# Autodesk Inventor assembly: Почти готово_CPY
(part 2 of 2)
- Жесткий:1 [WeldJoint]: Втулка под палец_CPY:1 ↔ Крейцкопф_CPY:1
- Жесткий:3 [WeldJoint]: Втулка палец шатун_CPY:1 ↔ Втулка под палец_CPY:2
- Жесткий:2 [WeldJoint]: Крейцкопф_CPY:1 ↔ Втулка под палец_CPY:2
- Жесткий:5 [WeldJoint]: Крейцкопф_CPY:1 ↔ Башмак_CPY:2
- С поворотом:1 [RevoluteJoint]: Втулка под палец_CPY:1 ↔ Палец_CPY:1
- Жесткий:7 [WeldJoint]: Палец_CPY:1 ↔ Стопорное кольцо_CPY:1
- Жесткий:6 [WeldJoint]: Палец_CPY:1 ↔ Стопорное кольцо_CPY:2
- Жесткий:14 [WeldJoint]: Гайка шток-поршень_CPY:1 ↔ Кольцо поршень-шток верх_CPY:1
- Жесткий:13 [WeldJoint]: Верхняя часть поршня_CPY:1 ↔ Кольцо поршень-шток верх_CPY:1
- Жесткий:9 [WeldJoint]: Верхняя часть поршня_CPY:1 ↔ Кольцо поршня_CPY:1
- С поворотом:3 [RevoluteJoint]: Корпус дросселя_CPY:1 ↔ Корпус сальника_CPY:1
- Жесткий:16 [WeldJoint]: Втулка_CPY:1 ↔ Крышка цилиндра 1_CPY:1
- Жесткий:70 [WeldJoint] (-2 mm): Фонарь_CPY:1 ↔ Крышка цилиндра 2_CPY:1
- Жесткий:12 [WeldJoint]: Кольцо поршень-шток низ_CPY:1 ↔ Нижняя часть поршня_CPY:1
- Жесткий:8 [WeldJoint]: Верхняя часть поршня_CPY:1 ↔ Нижняя часть поршня_CPY:1
- Жесткий:21 [WeldJoint]: Нижняя часть поршня_CPY:1 ↔ Опорное кольцо_CPY:1
- Жесткий:27 [WeldJoint]: Кольцо сальника_CPY:1 ↔ Пружина сальника_CPY:1
- Жесткий:79 [WeldJoint]: Крышка цилиндра 2_CPY:1 ↔ Цилиндр2_CPY:1
- Жесткий:23 [WeldJoint] (1 mm): Крышка стакана_CPY:1 ↔ Цилиндр2_CPY:1
- Жесткий:15 [WeldJoint]: Втулка_CPY:1 ↔ Цилиндр2_CPY:1
- Жесткий:11 [WeldJoint]: Нижняя часть поршня_CPY:1 ↔ Кольцо поршня_CPY:2
- Цилиндрический:1 [CylindricalJoint]: Втулка_CPY:1 ↔ Кольцо поршня_CPY:3
- Жесткий:10 [WeldJoint]: Нижняя часть поршня_CPY:1 ↔ Кольцо поршня_CPY:3
- Жесткий:80 [WeldJoint] (-2 mm): Цилиндр2_CPY:1 ↔ Клапан1_CPY:1
- Жесткий:18 [WeldJoint]: Цилиндр2_CPY:1 ↔ Прокладка клапана_CPY:1
- Жесткий:81 [WeldJoint] (-22 mm): Цилиндр2_CPY:1 ↔ Стакан1_CPY:1
- Жесткий:20 [WeldJoint]: Верхняя часть поршня_CPY:1 ↔ Опорное кольцо_CPY:2
- Жесткий:26 [WeldJoint]: Корпус дросселя_CPY:1 ↔ Дроссельное кольцо_CPY:1
- Жесткий:25 [WeldJoint] (2 mm): Пружина дросселя_CPY:1 ↔ Дроссельное кольцо_CPY:1
- Жесткий:32 [WeldJoint]: Корпус сальника_CPY:1 ↔ Кольцо сальника_CPY:2
- Жесткий:31 [WeldJoint]: Кольцо сальника_CPY:1 ↔ Кольцо сальника_CPY:2
- Жесткий:28 [WeldJoint]: Кольцо сальника_CPY:2 ↔ Пружина сальника_CPY:2
- Жесткий:30 [WeldJoint]: Кольцо сальника_CPY:1 ↔ Кольцо сальника_CPY:3
- Жесткий:29 [WeldJoint]: Кольцо сальника_CPY:3 ↔ Пружина сальника_CPY:3
- Жесткий:57 [WeldJoint]: Корпус сальника_CPY:1 ↔ Корпус сальника_CPY:2
- Жесткий:33 [WeldJoint]: Кольцо сальника_CPY:4 ↔ Пружина сальника_CPY:4
- Жесткий:38 [WeldJoint]: Корпус сальника_CPY:2 ↔ Кольцо сальника_CPY:5
- Жесткий:37 [WeldJoint]: Кольцо сальника_CPY:4 ↔ Кольцо сальника_CPY:5
- Жесткий:34 [WeldJoint]: Кольцо сальника_CPY:5 ↔ Пружина сальника_CPY:5
- Жесткий:36 [WeldJoint]: Кольцо сальника_CPY:4 ↔ Кольцо сальника_CPY:6
- Жесткий:35 [WeldJoint]: Кольцо сальника_CPY:6 ↔ Пружина сальника_CPY:6
- Жесткий:58 [WeldJoint]: Корпус сальника_CPY:2 ↔ Корпус сальника_CPY:3
- Жесткий:39 [WeldJoint]: Кольцо сальника_CPY:7 ↔ Пружина сальника_CPY:7
- Жесткий:44 [WeldJoint]: Корпус сальника_CPY:3 ↔ Кольцо сальника_CPY:8
- Жесткий:43 [WeldJoint]: Кольцо сальника_CPY:7 ↔ Кольцо сальника_CPY:8
- Жесткий:40 [WeldJoint]: Кольцо сальника_CPY:8 ↔ Пружина сальника_CPY:8
- Жесткий:42 [WeldJoint]: Кольцо сальника_CPY:7 ↔ Кольцо сальника_CPY:9
- Жесткий:41 [WeldJoint]: Кольцо сальника_CPY:9 ↔ Пружина сальника_CPY:9
- Жесткий:59 [WeldJoint]: Корпус сальника_CPY:3 ↔ Корпус сальника_CPY:4
- Жесткий:45 [WeldJoint]: Кольцо сальника_CPY:10 ↔ Пружина сальника_CPY:10
- Жесткий:50 [WeldJoint]: Корпус сальника_CPY:4 ↔ Кольцо сальника_CPY:11
- Жесткий:49 [WeldJoint]: Кольцо сальника_CPY:10 ↔ Кольцо сальника_CPY:11
- Жесткий:46 [WeldJoint]: Кольцо сальника_CPY:11 ↔ Пружина сальника_CPY:11
- Жесткий:48 [WeldJoint]: Кольцо сальника_CPY:10 ↔ Кольцо сальника_CPY:12
- Жесткий:47 [WeldJoint]: Кольцо сальника_CPY:12 ↔ Пружина сальника_CPY:12
- Жесткий:60 [WeldJoint]: Корпус сальника_CPY:4 ↔ Корпус сальника_CPY:5
- Жесткий:51 [WeldJoint]: Кольцо сальника_CPY:13 ↔ Пружина сальника_CPY:13
- Жесткий:56 [WeldJoint]: Корпус сальника_CPY:5 ↔ Кольцо сальника_CPY:14
- Жесткий:55 [WeldJoint]: Кольцо сальника_CPY:13 ↔ Кольцо сальника_CPY:14
- Жесткий:52 [WeldJoint]: Кольцо сальника_CPY:14 ↔ Пружина сальника_CPY:14
- Жесткий:54 [WeldJoint]: Кольцо сальника_CPY:13 ↔ Кольцо сальника_CPY:15
- Жесткий:53 [WeldJoint]: Кольцо сальника_CPY:15 ↔ Пружина сальника_CPY:15
- Жесткий:62 [WeldJoint] (-1 mm): Корпус дросселя_CPY:1 ↔ Уплотнительное кольцо_CPY:1
- Жесткий:61 [WeldJoint] (1 mm): Крышка цилиндра 2_CPY:1 ↔ Уплотнительное кольцо_CPY:1
- Жесткий:63 [WeldJoint]: Кольцо сальника_CPY:16 ↔ Пружина сальника_CPY:16
- Жесткий:67 [WeldJoint]: Кольцо сальника_CPY:16 ↔ Кольцо сальника_CPY:17
- Жесткий:64 [WeldJoint]: Кольцо сальника_CPY:17 ↔ Пружина сальника_CPY:17
- Жесткий:66 [WeldJoint]: Кольцо сальника_CPY:16 ↔ Кольцо сальника_CPY:18
- Жесткий:65 [WeldJoint]: Кольцо сальника_CPY:18 ↔ Пружина сальника_CPY:18
- Жесткий:69 [WeldJoint]: Фонарь_CPY:1 ↔ Уплотнение фонарь_CPY:1
- Жесткий:77 [WeldJoint]: Корпус сальника_CPY:5 ↔ Корпус сальника_CPY:6
- Жесткий:71 [WeldJoint]: Кольцо сальника_CPY:19 ↔ Пружина сальника_CPY:19
- Жесткий:76 [WeldJoint]: Корпус сальника_CPY:6 ↔ Кольцо сальника_CPY:20
- Жесткий:75 [WeldJoint]: Кольцо сальника_CPY:19 ↔ Кольцо сальника_CPY:20
- Жесткий:72 [WeldJoint]: Кольцо сальника_CPY:20 ↔ Пружина сальника_CPY:20
- Жесткий:74 [WeldJoint]: Кольцо сальника_CPY:19 ↔ Кольцо сальника_CPY:21
- Жесткий:73 [WeldJoint]: Кольцо сальника_CPY:21 ↔ Пружина сальника_CPY:21
- Жесткий:78 [WeldJoint] (3 mm): Крышка цилиндра 2_CPY:1 ↔ Крышка сальников_CPY:1
- Жесткий:95 [WeldJoint]: Корпус сальника перегородка 1_CPY:1 ↔ Крышка перегородки11_CPY:1
- Жесткий:94 [WeldJoint]: Фонарь_CPY:1 ↔ Крышка перегородки11_CPY:1
- Жесткий:96 [WeldJoint]: Корпус сальника перегородка 1_CPY:1 ↔ Крышка перегородки12_CPY:1
- Жесткий:104 [WeldJoint]: Корпус маслосъемника_CPY:1 ↔ Крышка перегородки21_CPY:1
- Жесткий:103 [WeldJoint]: Кольцо сальника_CPY:17 ↔ Крышка перегородки21_CPY:1
- Жесткий:98 [WeldJoint]: Фонарь_CPY:1 ↔ Крышка перегородки21_CPY:1
- Жесткий:105 [WeldJoint]: Крышка перегородки21_CPY:1 ↔ Крышка перегородки22_CPY:1
- Жесткий:99 [WeldJoint] (-1 mm): Маслосъемная пружина_CPY:1 ↔ Маслосъемное кольцо_CPY:1
- Жесткий:97 [WeldJoint]: Фонарь_CPY:1 ↔ Придав перегородки1_CPY:1
- Жесткий:82 [WeldJoint]: Кольцо сальника_CPY:22 ↔ Пружина сальника_CPY:22
- Жесткий:87 [WeldJoint]: Корпус сальника перегородка 1_CPY:1 ↔ Кольцо сальника_CPY:23
- Жесткий:86 [WeldJoint]: Кольцо сальника_CPY:22 ↔ Кольцо сальника_CPY:23
- Жесткий:83 [WeldJoint]: Кольцо сальника_CPY:23 ↔ Пружина сальника_CPY:23
- Жесткий:85 [WeldJoint]: Кольцо сальника_CPY:22 ↔ Кольцо сальника_CPY:24
- Жесткий:84 [WeldJoint]: Кольцо сальника_CPY:24 ↔ Пружина сальника_CPY:24
- Жесткий:88 [WeldJoint]: Кольцо сальника_CPY:25 ↔ Пружина сальника_CPY:25
- Жесткий:93 [WeldJoint]: Корпус сальника перегородка 1_CPY:1 ↔ Кольцо сальника_CPY:26
- Жесткий:92 [WeldJoint]: Кольцо сальника_CPY:25 ↔ Кольцо сальника_CPY:26
- Жесткий:89 [WeldJoint]: Кольцо сальника_CPY:26 ↔ Пружина сальника_CPY:26
- Жесткий:91 [WeldJoint]: Кольцо сальника_CPY:25 ↔ Кольцо сальника_CPY:27
- Жесткий:90 [WeldJoint]: Кольцо сальника_CPY:27 ↔ Пружина сальника_CPY:27
- Жесткий:102 [WeldJoint]: Корпус маслосъемника_CPY:1 ↔ Маслосъемное кольцо_CPY:2
- Жесткий:101 [WeldJoint]: Маслосъемное кольцо_CPY:1 ↔ Маслосъемное кольцо_CPY:2
- Жесткий:100 [WeldJoint] (-1 mm): Маслосъемная пружина_CPY:2 ↔ Маслосъемное кольцо_CPY:2
- Жесткий:106 [WeldJoint]: Фонарь_CPY:1 ↔ Придав перегородки1_CPY:2
- Жесткий:110 [WeldJoint] (-3 mm): Гайка шток_CPY:1 ↔ Шток_CPY:1
- Жесткий:107 [WeldJoint] (4.75 mm): Гайка шток-поршень_CPY:1 ↔ Шток_CPY:1
- Жесткий:207 [WeldJoint]: Фланецгайка_CPY:1 ↔ Прокладка крейцкопф_CPY:1
- Жесткий:206 [WeldJoint]: Крейцкопф_CPY:1 ↔ Прокладка крейцкопф_CPY:1
- Жесткий:112 [WeldJoint]: Крышка цилиндра 1_CPY:1 ↔ Шайба  ГОСТ 11371-78 25:1
- Жесткий:113 [WeldJoint] (-8.75 mm): Шпилька ГОСТ 22038-76 M24-6g×70:1 ↔ Гайка ГОСТ 15524-70 M24:1
- Жесткий:111 [WeldJoint]: Цилиндр2_CPY:1 ↔ Шпилька ГОСТ 22038-76 M24-6g×70:1
- Жесткий:114 [WeldJoint] (-8.75 mm): Шпилька ГОСТ 22038-76 M24-6g×70:2 ↔ Гайка ГОСТ 15524-70 M24:2
- Жесткий:116 [WeldJoint] (-2 mm): Цилиндр2_CPY:1 ↔ Клапан1_CPY:2
- Жесткий:115 [WeldJoint]: Цилиндр2_CPY:1 ↔ Прокладка клапана_CPY:2
- Жесткий:117 [WeldJoint] (-22 mm): Цилиндр2_CPY:1 ↔ Стакан1_CPY:2
- Жесткий:118 [WeldJoint] (1 mm): Цилиндр2_CPY:1 ↔ Крышка стакана_CPY:2
- Жесткий:119 [WeldJoint] (-1 mm): Цилиндр2_CPY:1 ↔ Шпилька ГОСТ 22034-76 M20-6g×50:1
- Жесткий:121 [WeldJoint] (-2.5 mm): Гайка ГОСТ 15521-70 M20:1 ↔ Шпилька ГОСТ 22034-76 M20-6g×50:1
- Жесткий:120 [WeldJoint] (-20 mm): Шпилька ГОСТ 22034-76 M20-6g×50:1 ↔ Шайба ГОСТ 10450-78 19:1
- Жесткий:122 [WeldJoint]: Цилиндр2_CPY:1 ↔ Шпилька ГОСТ 22034-76 M20-6g×50:2
- Жесткий:124 [WeldJoint] (-2.25 mm): Шпилька ГОСТ 22034-76 M20-6g×50:2 ↔ Гайка ГОСТ 15521-70 M20:2
- Жесткий:123 [WeldJoint] (-20 mm): Шпилька ГОСТ 22034-76 M20-6g×50:2 ↔ Шайба ГОСТ 10450-78 19:2
- Жесткий:127 [WeldJoint] (-2 mm): Фонарь_CPY:1 ↔ Гайка ГОСТ 15524-70 M20:1
- Жесткий:126 [WeldJoint] (-32 mm): Шпилька ГОСТ 22038-76 M20-6g×85:1 ↔ Шайба ГОСТ 10450-78 21:1
- Жесткий:125 [WeldJoint]: Крышка цилиндра 2_CPY:1 ↔ Шпилька ГОСТ 22038-76 M20-6g×85:1
- Жесткий:130 [WeldJoint]: Крышка перегородки22_CPY:1 ↔ Шайба  ГОСТ 11371-78 13:2
- Жесткий:134 [WeldJoint]: Придав перегородки1_CPY:1 ↔ Шайба  ГОСТ 11371-78 13:4
- Жесткий:128 [WeldJoint]: Крышка перегородки12_CPY:1 ↔ Шайба  ГОСТ 11371-78 13:1
- Жесткий:135 [WeldJoint]: Шайба  ГОСТ 11371-78 13:4 ↔ Винт ГОСТ 11738-84 M 10x25:2
- Жесткий:133 [WeldJoint]: Винт ГОСТ 11738-84 M 10x25:1 ↔ Шайба  ГОСТ 11371-78 13:3
- Жесткий:132 [WeldJoint]: Придав перегородки1_CPY:2 ↔ Шайба  ГОСТ 11371-78 13:3
- Жесткий:129 [WeldJoint]: Винт ГОСТ 11738-84 M 10x35:1 ↔ Шайба  ГОСТ 11371-78 13:1
- Жесткий:131 [WeldJoint]: Винт ГОСТ 11738-84 M 10x30:1 ↔ Шайба  ГОСТ 11371-78 13:2
- Жесткий:138 [WeldJoint] (-38 mm): Шпилька ГОСТ 22038-76 M24-6g×80:1 ↔ Гайка ГОСТ 15524-70 M24:18
- Жесткий:137 [WeldJoint] (-38 mm): Шпилька ГОСТ 22038-76 M24-6g×80:1 ↔ Шайба  ГОСТ 11371-78 28:1
- Жесткий:140 [WeldJoint] (-38 mm): Шпилька ГОСТ 22038-76 M24-6g×80:2 ↔ Гайка ГОСТ 15524-70 M24:19
- Жесткий:163 [WeldJoint]: Фонарь_CPY:1 ↔ Шайба  ГОСТ 11371-78 28:2
- Жесткий:139 [WeldJoint] (-38 mm): Шпилька ГОСТ 22038-76 M24-6g×80:2 ↔ Шайба  ГОСТ 11371-78 28:2
- Жесткий:142 [WeldJoint] (-38 mm): Шпилька ГОСТ 22038-76 M24-6g×80:3 ↔ Гайка ГОСТ 15524-70 M24:20
- Жесткий:165 [WeldJoint]: Фонарь_CPY:1 ↔ Шайба  ГОСТ 11371-78 28:3
- Жесткий:141 [WeldJoint] (-38 mm): Шпилька ГОСТ 22038-76 M24-6g×80:3 ↔ Шайба  ГОСТ 11371-78 28:3
- Жесткий:144 [WeldJoint] (-38 mm): Шпилька ГОСТ 22038-76 M24-6g×80:4 ↔ Гайка ГОСТ 15524-70 M24:21
- Жесткий:166 [WeldJoint]: Фонарь_CPY:1 ↔ Шайба  ГОСТ 11371-78 28:4
- Жесткий:143 [WeldJoint] (-38 mm): Шпилька ГОСТ 22038-76 M24-6g×80:4 ↔ Шайба  ГОСТ 11371-78 28:4
- Жесткий:146 [WeldJoint] (-38 mm): Шпилька ГОСТ 22038-76 M24-6g×80:5 ↔ Гайка ГОСТ 15524-70 M24:22
- Жесткий:164 [WeldJoint]: Фонарь_CPY:1 ↔ Шайба  ГОСТ 11371-78 28:5
- Жесткий:145 [WeldJoint] (-38 mm): Шпилька ГОСТ 22038-76 M24-6g×80:5 ↔ Шайба  ГОСТ 11371-78 28:5
- Жесткий:148 [WeldJoint] (-38 mm): Шпилька ГОСТ 22038-76 M24-6g×80:6 ↔ Гайка ГОСТ 15524-70 M24:23
- Жесткий:171 [WeldJoint]: Фонарь_CPY:1 ↔ Шайба  ГОСТ 11371-78 28:6
- Жесткий:147 [WeldJoint] (-38 mm): Шпилька ГОСТ 22038-76 M24-6g×80:6 ↔ Шайба  ГОСТ 11371-78 28:6
- Жесткий:150 [WeldJoint] (-38 mm): Шпилька ГОСТ 22038-76 M24-6g×80:7 ↔ Гайка ГОСТ 15524-70 M24:24
- Жесткий:173 [WeldJoint]: Фонарь_CPY:1 ↔ Шайба  ГОСТ 11371-78 28:7
- Жесткий:149 [WeldJoint] (-38 mm): Шпилька ГОСТ 22038-76 M24-6g×80:7 ↔ Шайба  ГОСТ 11371-78 28:7
- Жесткий:152 [WeldJoint] (-38 mm): Шпилька ГОСТ 22038-76 M24-6g×80:8 ↔ Гайка ГОСТ 15524-70 M24:25
- Жесткий:174 [WeldJoint]: Фонарь_CPY:1 ↔ Шайба  ГОСТ 11371-78 28:8
- Жесткий:151 [WeldJoint] (-38 mm): Шпилька ГОСТ 22038-76 M24-6g×80:8 ↔ Шайба  ГОСТ 11371-78 28:8
- Жесткий:154 [WeldJoint] (-38 mm): Шпилька ГОСТ 22038-76 M24-6g×80:9 ↔ Гайка ГОСТ 15524-70 M24:26
- Жесткий:172 [WeldJoint]: Фонарь_CPY:1 ↔ Шайба  ГОСТ 11371-78 28:9
- Жесткий:153 [WeldJoint] (-38 mm): Шпилька ГОСТ 22038-76 M24-6g×80:9 ↔ Шайба  ГОСТ 11371-78 28:9
- Жесткий:156 [WeldJoint] (-38 mm): Шпилька ГОСТ 22038-76 M24-6g×80:10 ↔ Гайка ГОСТ 15524-70 M24:27
- Жесткий:169 [WeldJoint]: Фонарь_CPY:1 ↔ Шайба  ГОСТ 11371-78 28:10
- Жесткий:155 [WeldJoint] (-38 mm): Шпилька ГОСТ 22038-76 M24-6g×80:10 ↔ Шайба  ГОСТ 11371-78 28:10
- Жесткий:158 [WeldJoint] (-38 mm): Шпилька ГОСТ 22038-76 M24-6g×80:11 ↔ Гайка ГОСТ 15524-70 M24:28
- Жесткий:167 [WeldJoint]: Фонарь_CPY:1 ↔ Шайба  ГОСТ 11371-78 28:11
- Жесткий:157 [WeldJoint] (-38 mm): Шпилька ГОСТ 22038-76 M24-6g×80:11 ↔ Шайба  ГОСТ 11371-78 28:11
- Жесткий:160 [WeldJoint] (-38 mm): Шпилька ГОСТ 22038-76 M24-6g×80:12 ↔ Гайка ГОСТ 15524-70 M24:29
- Жесткий:170 [WeldJoint]: Фонарь_CPY:1 ↔ Шайба  ГОСТ 11371-78 28:12
- Жесткий:159 [WeldJoint] (-38 mm): Шпилька ГОСТ 22038-76 M24-6g×80:12 ↔ Шайба  ГОСТ 11371-78 28:12
- Жесткий:162 [WeldJoint] (-38 mm): Шпилька ГОСТ 22038-76 M24-6g×80:13 ↔ Гайка ГОСТ 15524-70 M24:30
- Жесткий:168 [WeldJoint]: Фонарь_CPY:1 ↔ Шайба  ГОСТ 11371-78 28:13
- Жесткий:161 [WeldJoint] (-38 mm): Шпилька ГОСТ 22038-76 M24-6g×80:13 ↔ Шайба  ГОСТ 11371-78 28:13
- Жесткий:176 [WeldJoint] (-38 mm): Шпилька ГОСТ 22038-76 M24-6g×80:14 ↔ Гайка ГОСТ 15524-70 M24:31
- Жесткий:192 [WeldJoint]: Фонарь_CPY:1 ↔ Шайба  ГОСТ 11371-78 28:14
- Жесткий:175 [WeldJoint] (-38 mm): Шпилька ГОСТ 22038-76 M24-6g×80:14 ↔ Шайба  ГОСТ 11371-78 28:14
- Жесткий:178 [WeldJoint] (-38 mm): Шпилька ГОСТ 22038-76 M24-6g×80:15 ↔ Гайка ГОСТ 15524-70 M24:32
- Жесткий:197 [WeldJoint]: Фонарь_CPY:1 ↔ Шайба  ГОСТ 11371-78 28:15
- Жесткий:177 [WeldJoint] (-38 mm): Шпилька ГОСТ 22038-76 M24-6g×80:15 ↔ Шайба  ГОСТ 11371-78 28:15
- Жесткий:180 [WeldJoint] (-38 mm): Шпилька ГОСТ 22038-76 M24-6g×80:16 ↔ Гайка ГОСТ 15524-70 M24:33
- Жесткий:191 [WeldJoint]: Фонарь_CPY:1 ↔ Шайба  ГОСТ 11371-78 28:16
- Жесткий:179 [WeldJoint] (-38 mm): Шпилька ГОСТ 22038-76 M24-6g×80:16 ↔ Шайба  ГОСТ 11371-78 28:16
- Жесткий:184 [WeldJoint] (-38 mm): Шпилька ГОСТ 22038-76 M24-6g×80:17 ↔ Гайка ГОСТ 15524-70 M24:34
- Жесткий:196 [WeldJoint]: Фонарь_CPY:1 ↔ Шайба  ГОСТ 11371-78 28:17
- Жесткий:183 [WeldJoint] (-38 mm): Шпилька ГОСТ 22038-76 M24-6g×80:17 ↔ Шайба  ГОСТ 11371-78 28:17
- Жесткий:186 [WeldJoint] (-38 mm): Шпилька ГОСТ 22038-76 M24-6g×80:18 ↔ Гайка ГОСТ 15524-70 M24:35
- Жесткий:194 [WeldJoint]: Фонарь_CPY:1 ↔ Шайба  ГОСТ 11371-78 28:18
- Жесткий:185 [WeldJoint] (-38 mm): Шпилька ГОСТ 22038-76 M24-6g×80:18 ↔ Шайба  ГОСТ 11371-78 28:18
- Жесткий:188 [WeldJoint] (-38 mm): Шпилька ГОСТ 22038-76 M24-6g×80:19 ↔ Гайка ГОСТ 15524-70 M24:36
- Жесткий:193 [WeldJoint]: Фонарь_CPY:1 ↔ Шайба  ГОСТ 11371-78 28:19
- Жесткий:187 [WeldJoint] (-38 mm): Шпилька ГОСТ 22038-76 M24-6g×80:19 ↔ Шайба  ГОСТ 11371-78 28:19
- Жесткий:190 [WeldJoint] (-38 mm): Шпилька ГОСТ 22038-76 M24-6g×80:20 ↔ Гайка ГОСТ 15524-70 M24:37
- Жесткий:195 [WeldJoint]: Фонарь_CPY:1 ↔ Шайба  ГОСТ 11371-78 28:20
- Жесткий:189 [WeldJoint] (-38 mm): Шпилька ГОСТ 22038-76 M24-6g×80:20 ↔ Шайба  ГОСТ 11371-78 28:20
- Жесткий:198 [WeldJoint] (-2.5 mm): Гайка ГОСТ 15521-70 M20:3 ↔ Шпилька ГОСТ 22034-76 M20-6g×50:3
- Жесткий:199 [WeldJoint] (-20 mm): Шпилька ГОСТ 22034-76 M20-6g×50:3 ↔ Шайба ГОСТ 10450-78 19:3
- Жесткий:200 [WeldJoint] (-2.25 mm): Шпилька ГОСТ 22034-76 M20-6g×50:4 ↔ Гайка ГОСТ 15521-70 M20:4
- Жесткий:201 [WeldJoint] (-20 mm): Шпилька ГОСТ 22034-76 M20-6g×50:4 ↔ Шайба ГОСТ 10450-78 19:4
- Жесткий:208 [WeldJoint]: Крейцкопф_CPY:1 ↔ Шпилька ГОСТ 22038-76 M20-6g×85:2
- Жесткий:209 [WeldJoint]: Крейцкопф_CPY:1 ↔ Шпилька ГОСТ 22038-76 M20-6g×85:3
- Жесткий:211 [WeldJoint] (-26 mm): Шпилька ГОСТ 22038-76 M20-6g×85:2 ↔ Гайка ГОСТ 15524-70 M20:2
- Жесткий:210 [WeldJoint] (-26 mm): Шпилька ГОСТ 22038-76 M20-6g×85:2 ↔ Шайба  ГОСТ 11371-78 23:1
- Жесткий:213 [WeldJoint] (-2 mm): Шпилька ГОСТ 22038-76 M20-6g×85:3 ↔ Гайка ГОСТ 15524-70 M20:3
- Жесткий:212 [WeldJoint] (-26 mm): Шпилька ГОСТ 22038-76 M20-6g×85:3 ↔ Шайба  ГОСТ 11371-78 23:2
- Жесткий:404 [WeldJoint] (298.75 mm): Шток_CPY:1 ↔ Маслоотражательное кольцо_CPY:1
- Заподлицо:9 [Flush]: Фонарь_CPY:1 ↔ Крышка фонаря 1:1
- Заподлицо:10 [Flush]: Фонарь_CPY:1 ↔ Крышка фонаря 1:1
- Заподлицо:11 [Flush]: Фонарь_CPY:1 ↔ Крышка фонаря 2:1
- Заподлицо:12 [Flush]: Фонарь_CPY:1 ↔ Крышка фонаря 2:1
- Жесткий:395 [WeldJoint]: Крышка фонаря 1:1 ↔ Болт ГОСТ Р 50274-92 M8-6g×16-F:101
- Жесткий:396 [WeldJoint]: Крышка фонаря 1:1 ↔ Болт ГОСТ Р 50274-92 M8-6g×16-F:105
- Жесткий:397 [WeldJoint]: Крышка фонаря 1:1 ↔ Болт ГОСТ Р 50274-92 M8-6g×16-F:104
- Жесткий:398 [WeldJoint]: Крышка фонаря 1:1 ↔ Болт ГОСТ Р 50274-92 M8-6g×16-F:106
- Жесткий:399 [WeldJoint]: Крышка фонаря 1:1 ↔ Болт ГОСТ Р 50274-92 M8-6g×16-F:119
- Жесткий:400 [WeldJoint]: Крышка фонаря 1:1 ↔ Болт ГОСТ Р 50274-92 M8-6g×16-F:65
- Жесткий:401 [WeldJoint]: Крышка фонаря 1:1 ↔ Болт ГОСТ Р 50274-92 M8-6g×16-F:123
- Жесткий:402 [WeldJoint]: Крышка фонаря 1:1 ↔ Болт ГОСТ Р 50274-92 M8-6g×16-F:107
- Жесткий:403 [WeldJoint]: Крышка фонаря 1:1 ↔ Болт ГОСТ Р 50274-92 M8-6g×16-F:110
- Жесткий:404 [WeldJoint]: Крышка фонаря 1:1 ↔ Болт ГОСТ Р 50274-92 M8-6g×16-F:108
- Жесткий:405 [WeldJoint]: Крышка фонаря 1:1 ↔ Болт ГОСТ Р 50274-92 M8-6g×16-F:114
- Жесткий:406 [WeldJoint]: Крышка фонаря 1:1 ↔ Болт ГОСТ Р 50274-92 M8-6g×16-F:102
- С поворотом:3 [RevoluteJoint]: Крышка фонаря 2:1 ↔ Болт ГОСТ Р 50274-92 M8-6g×16-F:69
- С поворотом:4 [RevoluteJoint]: Крышка фонаря 2:1 ↔ Болт ГОСТ Р 50274-92 M8-6g×16-F:70
- С поворотом:5 [RevoluteJoint]: Крышка фонаря 2:1 ↔ Болт ГОСТ Р 50274-92 M8-6g×16-F:83
- Жесткий:407 [WeldJoint]: Крышка фонаря 2:1 ↔ Болт ГОСТ Р 50274-92 M8-6g×16-F:95
- Жесткий:408 [WeldJoint]: Крышка фонаря 2:1 ↔ Болт ГОСТ Р 50274-92 M8-6g×16-F:92
- Жесткий:409 [WeldJoint]: Крышка фонаря 2:1 ↔ Болт ГОСТ Р 50274-92 M8-6g×16-F:87
- Жесткий:410 [WeldJoint]: Крышка фонаря 2:1 ↔ Болт ГОСТ Р 50274-92 M8-6g×16-F:71
- Жесткий:411 [WeldJoint]: Крышка фонаря 2:1 ↔ Болт ГОСТ Р 50274-92 M8-6g×16-F:115
- Жесткий:412 [WeldJoint]: Крышка фонаря 2:1 ↔ Болт ГОСТ Р 50274-92 M8-6g×16-F:124
- Жесткий:413 [WeldJoint]: Крышка фонаря 2:1 ↔ Болт ГОСТ Р 50274-92 M8-6g×16-F:128
- Жесткий:414 [WeldJoint]: Крышка фонаря 2:1 ↔ Болт ГОСТ Р 50274-92 M8-6g×16-F:77
- Жесткий:415 [WeldJoint]: Крышка фонаря 2:1 ↔ Болт ГОСТ Р 50274-92 M8-6g×16-F:74
- Жесткий:416 [WeldJoint]: Крышка фонаря 2:1 ↔ Болт ГОСТ Р 50274-92 M8-6g×16-F:72
- Жесткий:417 [WeldJoint]: Крышка фонаря 2:1 ↔ Болт ГОСТ Р 50274-92 M8-6g×16-F:78
- Жесткий:418 [WeldJoint]: Крышка фонаря 2:1 ↔ Болт ГОСТ Р 50274-92 M8-6g×16-F:132
- Жесткий:419 [WeldJoint]: Крышка фонаря 2:1 ↔ Болт ГОСТ Р 50274-92 M8-6g×16-F:76
- Жесткий:420 [WeldJoint]: Крышка фонаря 2:1 ↔ Болт ГОСТ Р 50274-92 M8-6g×16-F:88
- Жесткий:421 [WeldJoint]: Крышка фонаря 2:1 ↔ Болт ГОСТ Р 50274-92 M8-6g×16-F:79
- Жесткий:422 [WeldJoint]: Крышка фонаря 2:1 ↔ Болт ГОСТ Р 50274-92 M8-6g×16-F:82
- Жесткий:423 [WeldJoint]: Крышка фонаря 2:1 ↔ Болт ГОСТ Р 50274-92 M8-6g×16-F:89
- Жесткий:424 [WeldJoint]: Крышка фонаря 2:1 ↔ Болт ГОСТ Р 50274-92 M8-6g×16-F:66
- Жесткий:425 [WeldJoint]: Крышка фонаря 2:1 ↔ Болт ГОСТ Р 50274-92 M8-6g×16-F:96
- Жесткий:426 [WeldJoint]: Крышка фонаря 2:1 ↔ Болт ГОСТ Р 50274-92 M8-6g×16-F:118
- Жесткий:427 [WeldJoint]: Крышка фонаря 2:1 ↔ Болт ГОСТ Р 50274-92 M8-6g×16-F:80
- Жесткий:428 [WeldJoint]: Крышка фонаря 1_MIR1:1 ↔ Болт ГОСТ Р 50274-92 M8-6g×16-F:133
- Жесткий:429 [WeldJoint]: Крышка фонаря 2_MIR1:1 ↔ Болт ГОСТ Р 50274-92 M8-6g×16-F:134
- С поворотом:6 [RevoluteJoint]: Крышка фонаря 2_MIR1:1 ↔ Болт ГОСТ Р 50274-92 M8-6g×16-F:135
- С поворотом:7 [RevoluteJoint]: Крышка фонаря 2_MIR1:1 ↔ Болт ГОСТ Р 50274-92 M8-6g×16-F:136
- Жесткий:430 [WeldJoint]: Крышка фонаря 2_MIR1:1 ↔ Болт ГОСТ Р 50274-92 M8-6g×16-F:137
- Жесткий:431 [WeldJoint]: Крышка фонаря 2_MIR1:1 ↔ Болт ГОСТ Р 50274-92 M8-6g×16-F:138
- Жесткий:432 [WeldJoint]: Крышка фонаря 2_MIR1:1 ↔ Болт ГОСТ Р 50274-92 M8-6g×16-F:139
- Жесткий:433 [WeldJoint]: Крышка фонаря 2_MIR1:1 ↔ Болт ГОСТ Р 50274-92 M8-6g×16-F:140
- Жесткий:434 [WeldJoint]: Крышка фонаря 2_MIR1:1 ↔ Болт ГОСТ Р 50274-92 M8-6g×16-F:141
- Жесткий:435 [WeldJoint]: Крышка фонаря 2_MIR1:1 ↔ Болт ГОСТ Р 50274-92 M8-6g×16-F:142
- Жесткий:436 [WeldJoint]: Крышка фонаря 2_MIR1:1 ↔ Болт ГОСТ Р 50274-92 M8-6g×16-F:143
- Жесткий:437 [WeldJoint]: Крышка фонаря 2_MIR1:1 ↔ Болт ГОСТ Р 50274-92 M8-6g×16-F:144
- Жесткий:438 [WeldJoint]: Крышка фонаря 2_MIR1:1 ↔ Болт ГОСТ Р 50274-92 M8-6g×16-F:145
- С поворотом:8 [RevoluteJoint]: Крышка фонаря 2_MIR1:1 ↔ Болт ГОСТ Р 50274-92 M8-6g×16-F:146
- Жесткий:439 [WeldJoint]: Крышка фонаря 2_MIR1:1 ↔ Болт ГОСТ Р 50274-92 M8-6g×16-F:147
- Жесткий:440 [WeldJoint]: Крышка фонаря 2_MIR1:1 ↔ Болт ГОСТ Р 50274-92 M8-6g×16-F:148
- Жесткий:441 [WeldJoint]: Крышка фонаря 2_MIR1:1 ↔ Болт ГОСТ Р 50274-92 M8-6g×16-F:149
- Жесткий:442 [WeldJoint]: Крышка фонаря 2_MIR1:1 ↔ Болт ГОСТ Р 50274-92 M8-6g×16-F:150
- Жесткий:443 [WeldJoint]: Крышка фонаря 2_MIR1:1 ↔ Болт ГОСТ Р 50274-92 M8-6g×16-F:151
- Жесткий:444 [WeldJoint]: Крышка фонаря 2_MIR1:1 ↔ Болт ГОСТ Р 50274-92 M8-6g×16-F:152
- Жесткий:445 [WeldJoint]: Крышка фонаря 1_MIR1:1 ↔ Болт ГОСТ Р 50274-92 M8-6g×16-F:153
- Жесткий:446 [WeldJoint]: Крышка фонаря 1_MIR1:1 ↔ Болт ГОСТ Р 50274-92 M8-6g×16-F:154
- Жесткий:447 [WeldJoint]: Крышка фонаря 1_MIR1:1 ↔ Болт ГОСТ Р 50274-92 M8-6g×16-F:155
- Жесткий:448 [WeldJoint]: Крышка фонаря 1_MIR1:1 ↔ Болт ГОСТ Р 50274-92 M8-6g×16-F:156
- Жесткий:449 [WeldJoint]: Крышка фонаря 1_MIR1:1 ↔ Болт ГОСТ Р 50274-92 M8-6g×16-F:157
- Жесткий:450 [WeldJoint]: Крышка фонаря 1_MIR1:1 ↔ Болт ГОСТ Р 50274-92 M8-6g×16-F:158
- Жесткий:451 [WeldJoint]: Крышка фонаря 1_MIR1:1 ↔ Болт ГОСТ Р 50274-92 M8-6g×16-F:159
- Жесткий:452 [WeldJoint]: Крышка фонаря 1_MIR1:1 ↔ Болт ГОСТ Р 50274-92 M8-6g×16-F:160
- Жесткий:453 [WeldJoint]: Крышка фонаря 1_MIR1:1 ↔ Болт ГОСТ Р 50274-92 M8-6g×16-F:161
- Жесткий:454 [WeldJoint]: Крышка фонаря 2_MIR1:1 ↔ Болт ГОСТ Р 50274-92 M8-6g×16-F:162
- Жесткий:455 [WeldJoint]: Крышка фонаря 2_MIR1:1 ↔ Болт ГОСТ Р 50274-92 M8-6g×16-F:163
- Жесткий:456 [WeldJoint]: Крышка фонаря 1_MIR1:1 ↔ Болт ГОСТ Р 50274-92 M8-6g×16-F:164
- Жесткий:457 [WeldJoint]: Крышка фонаря 1_MIR1:1 ↔ Болт ГОСТ Р 50274-92 M8-6g×16-F:165
- Жесткий:458 [WeldJoint]: Крышка фонаря 2_MIR1:1 ↔ Болт ГОСТ Р 50274-92 M8-6g×16-F:166
- Жесткий:459 [WeldJoint]: Крышка фонаря 2_MIR1:1 ↔ Болт ГОСТ Р 50274-92 M8-6g×16-F:167
- Жесткий:460 [WeldJoint]: Крышка фонаря 2_MIR1:1 ↔ Болт ГОСТ Р 50274-92 M8-6g×16-F:168
- Жесткий:461 [WeldJoint]: Цилиндр2_CPY:1 ↔ Деталь5_CPY:2
- Жесткий:462 [WeldJoint]: Болт ГОСТ Р 50274-92 M8-6g×16-F:175 ↔ Деталь6_CPY_MIR:1
- Жесткий:463 [WeldJoint]: Болт ГОСТ Р 50274-92 M8-6g×16-F:180 ↔ Деталь6_CPY_MIR:1
- Жесткий:464 [WeldJoint]: Болт ГОСТ Р 50274-92 M8-6g×16-F:174 ↔ Деталь6_CPY_MIR:1
- Жесткий:465 [WeldJoint]: Болт ГОСТ Р 50274-92 M8-6g×16-F:179 ↔ Деталь6_CPY_MIR:1
- Жесткий:466 [WeldJoint]: Болт ГОСТ Р 50274-92 M8-6g×16-F:178 ↔ Деталь6_CPY_MIR:1
- Жесткий:467 [WeldJoint]: Болт ГОСТ Р 50274-92 M8-6g×16-F:171 ↔ Деталь6_CPY_MIR:1
- Жесткий:468 [WeldJoint]: Болт ГОСТ Р 50274-92 M8-6g×16-F:192 ↔ Деталь6_CPY_MIR:1
- Жесткий:469 [WeldJoint]: Болт ГОСТ Р 50274-92 M8-6g×16-F:191 ↔ Деталь6_CPY_MIR:1
- Жесткий:470 [WeldJoint]: Болт ГОСТ Р 50274-92 M8-6g×16-F:190 ↔ Деталь6_CPY_MIR:1
- Жесткий:471 [WeldJoint]: Болт ГОСТ Р 50274-92 M8-6g×16-F:189 ↔ Деталь6_CPY_MIR:1
- Жесткий:472 [WeldJoint]: Болт ГОСТ Р 50274-92 M8-6g×16-F:188 ↔ Деталь6_CPY_MIR:1
- Жесткий:473 [WeldJoint]: Болт ГОСТ Р 50274-92 M8-6g×16-F:173 ↔ Деталь6_CPY_MIR:1
- Жесткий:474 [WeldJoint]: Болт ГОСТ Р 50274-92 M8-6g×16-F:172 ↔ Деталь6_CPY_MIR:1
- Жесткий:475 [WeldJoint]: Болт ГОСТ Р 50274-92 M8-6g×16-F:170 ↔ Деталь6_CPY_MIR:1
- Жесткий:476 [WeldJoint]: Болт ГОСТ Р 50274-92 M8-6g×16-F:187 ↔ Деталь6_CPY_MIR:1
- Жесткий:477 [WeldJoint]: Болт ГОСТ Р 50274-92 M8-6g×16-F:169 ↔ Деталь6_CPY_MIR:1
